# Autodesk Inventor assembly: ASSEMBLY_Main
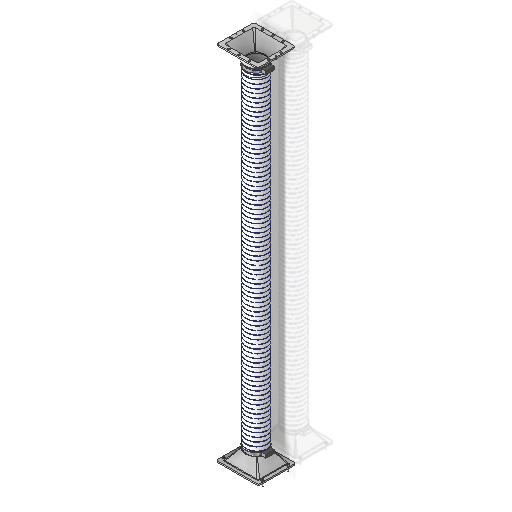
[picture p0: Inventor's stored thumbnail of the model, 512x512]
Saved by Autodesk Inventor 2025 (Build 290162010, 162A)
## iProperties
Created: 2024-10-12
Part Number: ASSEMBLY_Main
Document SubType Name: Assembly
Designer: User
Author: User
## Documents named in this file (9)
- D:\_ANDRZEJ_LACZEWSKI\_OTHER\MCAD\1_REV1\ASSEMBLY_MAIN_REVA\ASSEMBLY_Main.iam
- D:\_ANDRZEJ_LACZEWSKI\_OTHER\MCAD\1_REV1\ASSEMBLY_MAIN_REVA\3DP_PLA_Air_Purifier_60mm_Pipe_Mount.ipt
- D:\_ANDRZEJ_LACZEWSKI\_OTHER\MCAD\1_REV1\ASSEMBLY_MAIN_REVA\3DP_PLA_X1C_60mm_Pipe_Mount.ipt
- D:\_ANDRZEJ_LACZEWSKI\_OTHER\MCAD\1_REV1\__COTS_PARTS\COTS_GENERIC_6x3mm_Cylindricial_Neodymium_Magnet.ipt
- D:\_ANDRZEJ_LACZEWSKI\_OTHER\MCAD\1_REV1\__COTS_PARTS\COTS_GENERIC_60mm_PUR_Suction_Hose.ipt
- D:\_ANDRZEJ_LACZEWSKI\_OTHER\MCAD\1_REV1\__CONTENT_CENTER_PARTS\en-US\DIN 912\DIN 912 - M2,5 x 0,45 x 6 x 4,875.ipt
- D:\_ANDRZEJ_LACZEWSKI\_OTHER\MCAD\1_REV1\__CONTENT_CENTER_PARTS\en-US\DIN 125-2  A\DIN 125-2 - A 3,2A.ipt
- D:\_ANDRZEJ_LACZEWSKI\_OTHER\MCAD\1_REV1\__CONTENT_CENTER_PARTS\en-US\DIN 912\DIN 912 - M3 x 0,5 x 16 x 14,75.ipt
- D:\_ANDRZEJ_LACZEWSKI\_OTHER\MCAD\1_REV1\__COTS_PARTS\COTS_GENERIC_60mm_Hose_Clamp.ipt
## Components (25 placed, 8 different names)
1. 3DP_PLA_Air_Purifier_60mm_Pipe_Mount:1 — Mate:1, Angle:1, Mate:4, Mate:29, Mate:30, Mate:31, Mate:32, Mate:33, Mate:34, Mate:35, Mate:36, Flush:3
2. 3DP_PLA_X1C_60mm_Pipe_Mount:1 — Mate:2, Angle:1, Mate:3, Mate:5, Mate:6, Mate:7, Mate:8, Mate:9, Mate:10, Mate:11, Mate:12, Mate:13, Mate:14, Mate:15, Mate:16, Mate:17, Mate:18, Mate:19, Mate:20, Mate:21, Mate:22, Mate:23, Mate:24, Mate:25, Mate:26, Mate:27, Mate:28
3. COTS_GENERIC_6x3mm_Cylindricial_Neodymium_Magnet:1 — Mate:5, Mate:6
4. COTS_GENERIC_60mm_PUR_Suction_Hose:1 — Mate:1, Mate:2, Mate:3, Mate:4, Mate:37, Mate:38, Flush:1, Flush:2
5. COTS_GENERIC_6x3mm_Cylindricial_Neodymium_Magnet:2 — Mate:15, Mate:16
6. COTS_GENERIC_6x3mm_Cylindricial_Neodymium_Magnet:3 — Mate:14, Mate:17
7. COTS_GENERIC_6x3mm_Cylindricial_Neodymium_Magnet:4 — Mate:13, Mate:18
8. COTS_GENERIC_6x3mm_Cylindricial_Neodymium_Magnet:5 — Mate:12, Mate:19
9. COTS_GENERIC_6x3mm_Cylindricial_Neodymium_Magnet:6 — Mate:11, Mate:20
10. COTS_GENERIC_6x3mm_Cylindricial_Neodymium_Magnet:7 — Mate:10, Mate:21
11. COTS_GENERIC_6x3mm_Cylindricial_Neodymium_Magnet:8 — Mate:9, Mate:22
12. COTS_GENERIC_6x3mm_Cylindricial_Neodymium_Magnet:9 — Mate:8, Mate:23
13. COTS_GENERIC_6x3mm_Cylindricial_Neodymium_Magnet:10 — Mate:7, Mate:24
14. COTS_GENERIC_60mm_Hose_Clamp:1 — Mate:37, Flush:2
15. COTS_GENERIC_60mm_Hose_Clamp:2 — Mate:38, Flush:1
16. DIN 912 - replaced by DIN EN ISO 4762 M2,5 x 6:1 — Mate:25, Mate:26
17. DIN 912 - replaced by DIN EN ISO 4762 M2,5 x 6:2 — Mate:27, Mate:28
18. DIN 125-2 A A 3,2:1 — Mate:29, Mate:30, Insert:1
19. DIN 912 - replaced by DIN EN ISO 4762 M3 x 16:1 — Insert:1
20. DIN 125-2 A A 3,2:2 — Mate:31, Mate:32, Insert:2
21. DIN 125-2 A A 3,2:3 — Mate:33, Mate:34, Insert:3
22. DIN 125-2 A A 3,2:4 — Mate:35, Mate:36, Insert:4
23. DIN 912 - replaced by DIN EN ISO 4762 M3 x 16:2 — Insert:2
24. DIN 912 - replaced by DIN EN ISO 4762 M3 x 16:3 — Insert:3
25. DIN 912 - replaced by DIN EN ISO 4762 M3 x 16:4 — Insert:4
## Relationships (46: Mate 38, Insert 4, Flush 3, Angle 1)
- Mate:1: 3DP_PLA_Air_Purifier_60mm_Pipe_Mount:1 ↔ COTS_GENERIC_60mm_PUR_Suction_Hose:1
- Mate:2: 3DP_PLA_X1C_60mm_Pipe_Mount:1 ↔ COTS_GENERIC_60mm_PUR_Suction_Hose:1
- Angle:1 (0 deg): 3DP_PLA_Air_Purifier_60mm_Pipe_Mount:1 ↔ 3DP_PLA_X1C_60mm_Pipe_Mount:1
- Mate:3 (-25 mm): 3DP_PLA_X1C_60mm_Pipe_Mount:1 ↔ COTS_GENERIC_60mm_PUR_Suction_Hose:1
- Mate:4 (-25 mm): 3DP_PLA_Air_Purifier_60mm_Pipe_Mount:1 ↔ COTS_GENERIC_60mm_PUR_Suction_Hose:1
- Mate:5: 3DP_PLA_X1C_60mm_Pipe_Mount:1 ↔ COTS_GENERIC_6x3mm_Cylindricial_Neodymium_Magnet:1
- Mate:6: 3DP_PLA_X1C_60mm_Pipe_Mount:1 ↔ COTS_GENERIC_6x3mm_Cylindricial_Neodymium_Magnet:1
- Mate:7: 3DP_PLA_X1C_60mm_Pipe_Mount:1 ↔ COTS_GENERIC_6x3mm_Cylindricial_Neodymium_Magnet:10
- Mate:8: 3DP_PLA_X1C_60mm_Pipe_Mount:1 ↔ COTS_GENERIC_6x3mm_Cylindricial_Neodymium_Magnet:9
- Mate:9: 3DP_PLA_X1C_60mm_Pipe_Mount:1 ↔ COTS_GENERIC_6x3mm_Cylindricial_Neodymium_Magnet:8
- Mate:10: 3DP_PLA_X1C_60mm_Pipe_Mount:1 ↔ COTS_GENERIC_6x3mm_Cylindricial_Neodymium_Magnet:7
- Mate:11: 3DP_PLA_X1C_60mm_Pipe_Mount:1 ↔ COTS_GENERIC_6x3mm_Cylindricial_Neodymium_Magnet:6
- Mate:12: 3DP_PLA_X1C_60mm_Pipe_Mount:1 ↔ COTS_GENERIC_6x3mm_Cylindricial_Neodymium_Magnet:5
- Mate:13: 3DP_PLA_X1C_60mm_Pipe_Mount:1 ↔ COTS_GENERIC_6x3mm_Cylindricial_Neodymium_Magnet:4
- Mate:14: 3DP_PLA_X1C_60mm_Pipe_Mount:1 ↔ COTS_GENERIC_6x3mm_Cylindricial_Neodymium_Magnet:3
- Mate:15: 3DP_PLA_X1C_60mm_Pipe_Mount:1 ↔ COTS_GENERIC_6x3mm_Cylindricial_Neodymium_Magnet:2
- Mate:16: 3DP_PLA_X1C_60mm_Pipe_Mount:1 ↔ COTS_GENERIC_6x3mm_Cylindricial_Neodymium_Magnet:2
- Mate:17: 3DP_PLA_X1C_60mm_Pipe_Mount:1 ↔ COTS_GENERIC_6x3mm_Cylindricial_Neodymium_Magnet:3
- Mate:18: 3DP_PLA_X1C_60mm_Pipe_Mount:1 ↔ COTS_GENERIC_6x3mm_Cylindricial_Neodymium_Magnet:4
- Mate:19: 3DP_PLA_X1C_60mm_Pipe_Mount:1 ↔ COTS_GENERIC_6x3mm_Cylindricial_Neodymium_Magnet:5
- Mate:20: 3DP_PLA_X1C_60mm_Pipe_Mount:1 ↔ COTS_GENERIC_6x3mm_Cylindricial_Neodymium_Magnet:6
- Mate:21: 3DP_PLA_X1C_60mm_Pipe_Mount:1 ↔ COTS_GENERIC_6x3mm_Cylindricial_Neodymium_Magnet:7
- Mate:22: 3DP_PLA_X1C_60mm_Pipe_Mount:1 ↔ COTS_GENERIC_6x3mm_Cylindricial_Neodymium_Magnet:8
- Mate:23: 3DP_PLA_X1C_60mm_Pipe_Mount:1 ↔ COTS_GENERIC_6x3mm_Cylindricial_Neodymium_Magnet:9
- Mate:24: 3DP_PLA_X1C_60mm_Pipe_Mount:1 ↔ COTS_GENERIC_6x3mm_Cylindricial_Neodymium_Magnet:10
- Mate:25: 3DP_PLA_X1C_60mm_Pipe_Mount:1 ↔ DIN 912 - replaced by DIN EN ISO 4762 M2,5 x 6:1
- Mate:26: 3DP_PLA_X1C_60mm_Pipe_Mount:1 ↔ DIN 912 - replaced by DIN EN ISO 4762 M2,5 x 6:1
- Mate:27: 3DP_PLA_X1C_60mm_Pipe_Mount:1 ↔ DIN 912 - replaced by DIN EN ISO 4762 M2,5 x 6:2
- Mate:28: 3DP_PLA_X1C_60mm_Pipe_Mount:1 ↔ DIN 912 - replaced by DIN EN ISO 4762 M2,5 x 6:2
- Mate:29: 3DP_PLA_Air_Purifier_60mm_Pipe_Mount:1 ↔ DIN 125-2 A A 3,2:1
- Mate:30: 3DP_PLA_Air_Purifier_60mm_Pipe_Mount:1 ↔ DIN 125-2 A A 3,2:1
- Mate:31: 3DP_PLA_Air_Purifier_60mm_Pipe_Mount:1 ↔ DIN 125-2 A A 3,2:2
- Mate:32: 3DP_PLA_Air_Purifier_60mm_Pipe_Mount:1 ↔ DIN 125-2 A A 3,2:2
- Mate:33: 3DP_PLA_Air_Purifier_60mm_Pipe_Mount:1 ↔ DIN 125-2 A A 3,2:3
- Mate:34: 3DP_PLA_Air_Purifier_60mm_Pipe_Mount:1 ↔ DIN 125-2 A A 3,2:3
- Mate:35: 3DP_PLA_Air_Purifier_60mm_Pipe_Mount:1 ↔ DIN 125-2 A A 3,2:4
- Mate:36: 3DP_PLA_Air_Purifier_60mm_Pipe_Mount:1 ↔ DIN 125-2 A A 3,2:4
- Insert:1: DIN 125-2 A A 3,2:1 ↔ DIN 912 - replaced by DIN EN ISO 4762 M3 x 16:1
- Insert:2: DIN 125-2 A A 3,2:2 ↔ DIN 912 - replaced by DIN EN ISO 4762 M3 x 16:2
- Insert:3: DIN 125-2 A A 3,2:3 ↔ DIN 912 - replaced by DIN EN ISO 4762 M3 x 16:3
- Insert:4: DIN 125-2 A A 3,2:4 ↔ DIN 912 - replaced by DIN EN ISO 4762 M3 x 16:4
- Mate:37: COTS_GENERIC_60mm_PUR_Suction_Hose:1 ↔ COTS_GENERIC_60mm_Hose_Clamp:1
- Mate:38: COTS_GENERIC_60mm_PUR_Suction_Hose:1 ↔ COTS_GENERIC_60mm_Hose_Clamp:2
- Flush:1: COTS_GENERIC_60mm_PUR_Suction_Hose:1 ↔ COTS_GENERIC_60mm_Hose_Clamp:2
- Flush:2: COTS_GENERIC_60mm_PUR_Suction_Hose:1 ↔ COTS_GENERIC_60mm_Hose_Clamp:1
- Flush:3: 3DP_PLA_Air_Purifier_60mm_Pipe_Mount:1
